# Autodesk Inventor assembly: Ender
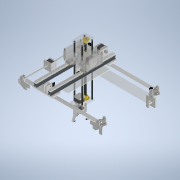
[picture p0: Inventor's stored thumbnail of the model, 180x180]
Saved by Autodesk Inventor 2022 (Build 260153000, 153)
## iProperties
Created: 2021-06-26
Part Number: Ender
Document SubType Name: Assembly
Designer: domin
Author: domin
## Documents named in this file (5)
- C:\Users\kaebi\OneDrive - mci4me.at\03_MCI Master\4.Semester_SS2022\Masterarbeit\Software\CAD_TeachingFactory\Ender.iam
- C:\Users\kaebi\OneDrive - mci4me.at\03_MCI Master\4.Semester_SS2022\Masterarbeit\Software\CAD_TeachingFactory\XAxis.iam
- C:\Users\kaebi\OneDrive - mci4me.at\03_MCI Master\4.Semester_SS2022\Masterarbeit\Software\CAD_TeachingFactory\YAxis.iam
- C:\Users\kaebi\OneDrive - mci4me.at\03_MCI Master\4.Semester_SS2022\Masterarbeit\Software\CAD_TeachingFactory\ZAxis.iam
- C:\Users\kaebi\OneDrive - mci4me.at\03_MCI Master\4.Semester_SS2022\Masterarbeit\Software\CAD_TeachingFactory\ZAxisRodsandGripper.iam
## Components (4 placed, 4 different names)
1. XAxis:1 [sub-assembly] — Flush:1, Flush:2, Flush:3, Slider:1
2. YAxis:1 [sub-assembly] — Slider:1, Slider:2
3. ZAxis:1 [sub-assembly] — Slider:2, Cylindrical:1, Angle:1
4. ZAxisRodsandGripper:1 [sub-assembly] — Cylindrical:1, Angle:1
## Relationships (7: Flush 3, TranslationJoint 2, CylindricalJoint 1, Angle 1)
- Flush:1: XAxis:1
- Flush:2: XAxis:1
- Flush:3: XAxis:1
- Slider:1 [TranslationJoint]: XAxis:1 ↔ YAxis:1
- Slider:2 [TranslationJoint]: YAxis:1 ↔ ZAxis:1
- Cylindrical:1: ZAxis:1 ↔ ZAxisRodsandGripper:1
- Angle:1 (0 deg): ZAxis:1 ↔ ZAxisRodsandGripper:1
